# Autodesk Inventor assembly: 脚右
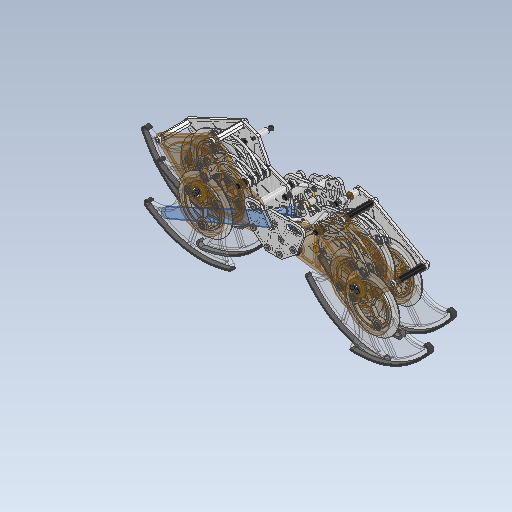
[picture p0: Inventor's stored thumbnail of the model, 512x512]
Saved by Autodesk Inventor 2020.2 (Build 242310000, 310)
## iProperties
Created: 2020-04-15
Part Number: 脚右
Document SubType Name: Assembly
Designer: aoyama
Mass: 557.301 g
Surface Area: 3848.31 cm^2
Volume: 258.765 cm^3
Density: 2.1537 g/cm^3
Author: aoyama
## Documents named in this file (17)
- C:\Users\aoyam\Desktop\SRDC_local\Inventor\二年機\Geminiβ\脚\脚右.iam
- C:\Users\aoyam\Desktop\SRDC_local\Inventor\二年機\Geminiβ\脚\脚四半.iam
- C:\Users\aoyam\Desktop\SRDC_local\Inventor\二年機\Geminiβ\脚\中間ユニット\中間ユニット.iam
- C:\Users\aoyam\Desktop\SRDC_local\Inventor\二年機\Geminiβ\汎用部品\オイレスFd6D8L3.ipt
- C:\Users\aoyam\Desktop\SRDC_local\Inventor\二年機\Geminiβ\脚\MIR達\MIRright脚四半.iam
- C:\Users\aoyam\Desktop\SRDC_local\Inventor\二年機\Geminiβ\汎用部品\スペーサー中空M3L8アルミ.ipt
- C:\Users\aoyam\Desktop\SRDC_local\Inventor\二年機\Geminiβ\汎用部品\ワッシャD7d3m0.5.ipt
- C:\Users\aoyam\Desktop\SRDC_local\Inventor\二年機\Geminiβ\汎用部品\スペーサーM3L8アルミ.ipt
- C:\Users\aoyam\Desktop\SRDC_local\Inventor\二年機\Geminiβ\汎用部品\ネジボタンM3L6.ipt
- C:\Users\aoyam\Desktop\SRDC_local\Inventor\二年機\Geminiβ\脚\ダンパーガード.ipt
- C:\Users\aoyam\Desktop\SRDC_local\Inventor\二年機\Geminiβ\汎用部品\スペーサー中空M3L12アルミ.ipt
- C:\Users\aoyam\Desktop\SRDC_local\Inventor\二年機\Geminiβ\汎用部品\ネジボタンM3L22.ipt
- C:\Users\aoyam\Desktop\SRDC_local\Inventor\二年機\Geminiβ\汎用部品\ナットナイロンM3.ipt
- C:\Users\aoyam\Desktop\SRDC_local\Inventor\二年機\Geminiβ\汎用部品\ネジボタンM3L8.ipt
- C:\Users\aoyam\Desktop\SRDC_local\Inventor\二年機\Geminiβ\汎用部品\ネジボタンM3L20.ipt
- C:\Users\aoyam\Desktop\SRDC_local\Inventor\二年機\Geminiβ\翼\MIRrightWingUnit2L.iam
- C:\Users\aoyam\Desktop\SRDC_local\Inventor\二年機\Geminiβ\汎用部品\ネジ皿M3L4.ipt
## Components (18 placed, 16 different names)
1. 脚四半:1 [sub-assembly] — 挿入:39, 挿入:47
2. 中間ユニット:1 [sub-assembly] — 挿入:13, 挿入:42, 挿入:43, 挿入:44, 挿入:45, 挿入:46, 挿入:47, 挿入:48, 挿入:49, 挿入:50
3. オイレスFd6D8L3:1 — 挿入:42
4. オイレスFd6D8L3:2 — 挿入:43
5. MIRright脚四半:1 [sub-assembly] — メイト:1, 挿入:40, 挿入:41, 挿入:48
6. ワッシャD7d3m0.5:1 — 挿入:5, 挿入:6
7. スペーサーM3L8アルミ:1 — 挿入:5, 挿入:41
8. スペーサー中空M3L8アルミ:1 — 挿入:6, 挿入:9
9. ネジボタンM3L6:1 — 挿入:40
10. ダンパーガード:1 — 挿入:9, メイト:1
11. スペーサー中空M3L12アルミ:1 — 挿入:12, 挿入:39
12. ネジボタンM3L22:1 — 挿入:12
13. ナットナイロンM3:1
14. ネジボタンM3L8:1 — 挿入:13
15. ネジボタンM3L20:1
16. MIRrightWingUnit2L:1 [sub-assembly] — 挿入:44, 挿入:45, 挿入:46
17. ネジ皿M3L4:1 — 挿入:49
18. ネジ皿M3L4:2 — 挿入:50
## Relationships (18: Insert 17, Mate 1)
- 挿入:5 [Insert]: ワッシャD7d3m0.5:1 ↔ スペーサーM3L8アルミ:1
- 挿入:6 [Insert] (5 mm): ワッシャD7d3m0.5:1 ↔ スペーサー中空M3L8アルミ:1
- 挿入:9 [Insert]: スペーサー中空M3L8アルミ:1 ↔ ダンパーガード:1
- メイト:1 [Mate]: MIRright脚四半:1 ↔ ダンパーガード:1
- 挿入:12 [Insert] (5 mm): スペーサー中空M3L12アルミ:1 ↔ ネジボタンM3L22:1
- 挿入:13 [Insert] (5 mm): 中間ユニット:1 ↔ ネジボタンM3L8:1
- 挿入:39 [Insert]: 脚四半:1 ↔ スペーサー中空M3L12アルミ:1
- 挿入:40 [Insert]: MIRright脚四半:1 ↔ ネジボタンM3L6:1
- 挿入:41 [Insert]: MIRright脚四半:1 ↔ スペーサーM3L8アルミ:1
- 挿入:42 [Insert]: 中間ユニット:1 ↔ オイレスFd6D8L3:1
- 挿入:43 [Insert]: 中間ユニット:1 ↔ オイレスFd6D8L3:2
- 挿入:44 [Insert]: 中間ユニット:1 ↔ MIRrightWingUnit2L:1
- 挿入:45 [Insert]: 中間ユニット:1 ↔ MIRrightWingUnit2L:1
- 挿入:46 [Insert]: 中間ユニット:1 ↔ MIRrightWingUnit2L:1
- 挿入:47 [Insert]: 脚四半:1 ↔ 中間ユニット:1
- 挿入:48 [Insert]: 中間ユニット:1 ↔ MIRright脚四半:1
- 挿入:49 [Insert]: 中間ユニット:1 ↔ ネジ皿M3L4:1
- 挿入:50 [Insert]: 中間ユニット:1 ↔ ネジ皿M3L4:2
